# Autodesk Inventor assembly: Ensamblaje1
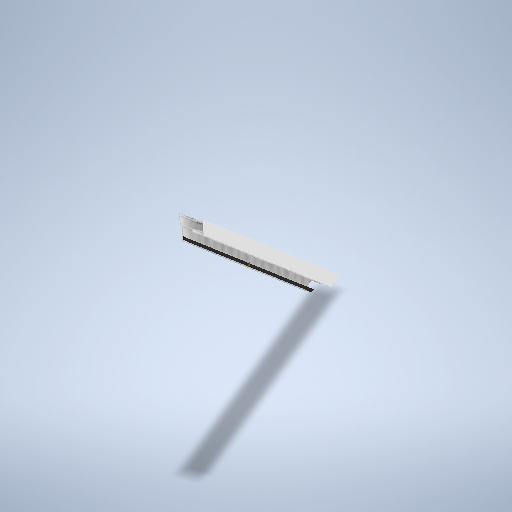
[picture p0: Inventor's stored thumbnail of the model, 512x512]
Saved by Autodesk Inventor 2025 (Build 290162000, 162)
## iProperties
Created: 2026-02-12
Part Number: Ensamblaje1
Document SubType Name: Assembly
Designer: Frank
Author: Frank
## Documents named in this file (3)
- D:\Inventor\Proyectos\MARQUTERIA DE ALUMINIO\MARCOS INTERIOR\Ensamblaje1.iam
- D:\Inventor\Proyectos\MARQUTERIA DE ALUMINIO\MARCOS INTERIOR\SP40-01 MARCO BATIENTE - PAÑO FIJO 800MM.ipt
- D:\Inventor\Proyectos\MARQUTERIA DE ALUMINIO\MARCOS INTERIOR\JUNTA DE GOMA 800MM.ipt
## Components (2 placed, 2 different names)
1. SP40-01 MARCO BATIENTE - PAÑO FIJO 800MM:1 — Coincidencia:1, Coincidencia:2, Coincidencia:3
2. JUNTA DE GOMA 800MM:1 — Coincidencia:1, Coincidencia:2, Coincidencia:3
## Relationships (3: Mate 3)
- Coincidencia:1 [Mate]: SP40-01 MARCO BATIENTE - PAÑO FIJO 800MM:1 ↔ JUNTA DE GOMA 800MM:1
- Coincidencia:2 [Mate]: SP40-01 MARCO BATIENTE - PAÑO FIJO 800MM:1 ↔ JUNTA DE GOMA 800MM:1
- Coincidencia:3 [Mate]: SP40-01 MARCO BATIENTE - PAÑO FIJO 800MM:1 ↔ JUNTA DE GOMA 800MM:1
